# Autodesk Inventor assembly: 3000_Sample Assembly_V2
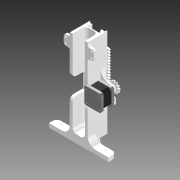
[picture p0: Inventor's stored thumbnail of the model, 180x180]
Saved by Autodesk Inventor 2021 (Build 250183000, 183)
## iProperties
Created: 2019-11-07
Part Number: 3000_Sample Assembly_V2
Document SubType Name: Assembly
Designer: RFLab
Author: RFLab
## Documents named in this file (7)
- C:\Users\RFLab\Documents\GitHub\MPS\Inventor Parts\MPSV2\6xxx_Sample Assembly\6000_Sample Assembly_V2.iam
- C:\Users\RFLab\Documents\GitHub\MPS\Inventor Parts\MPSV2\6xxx_Sample Assembly\61xx_Sample Rails\6101_Sample Rail Base_V2.ipt
- C:\Users\RFLab\Documents\GitHub\MPS\Inventor Parts\MPSV2\6xxx_Sample Assembly\61xx_Sample Rails\6102_Dovetail Slider_V2.ipt
- C:\Users\RFLab\Documents\GitHub\MPS\Inventor Parts\MPSV2\6xxx_Sample Assembly\62xx_ Motor and Driving\621x_Stepper Motor Parts\6211_Stepper Motor_V1.ipt
- C:\Users\RFLab\Documents\GitHub\MPS\Inventor Parts\MPSV2\6xxx_Sample Assembly\62xx_ Motor and Driving\622x_Motor Mechanical Connectors\6221_Motor Pinion_V3.ipt
- C:\Users\RFLab\Documents\GitHub\MPS\Inventor Parts\MPSV2\6xxx_Sample Assembly\61xx_Sample Rails\6104_Example Bulb_V1.ipt
- C:\Users\RFLab\Documents\GitHub\MPS\Inventor Parts\MPSV2\6xxx_Sample Assembly\61xx_Sample Rails\6103_Bulb Arm_V4.ipt
## Components (6 placed, 6 different names)
1. 6101_Sample Rail Base_V2:1 — Mate:1, Mate:2, Mate:13, Mate:14, Mate:15, Flush:3, Mate:17, Flush:4
2. 6102_Dovetail Slider_V2:1 — Mate:1, Mate:2, Mate:23, Flush:5, Mate:24
3. 6211_Stepper Motor_V1:1 — Flush:3, Mate:17, Flush:4, Rotational:1
4. Spur Gear1:2 — Rotational:1
5. 6104_Example Bulb_V1:1 — Mate:25, Mate:26
6. 6103_Bulb Arm_V4:1 — Mate:23, Flush:5, Mate:24, Mate:25, Mate:26
## Relationships (14: Mate 10, Flush 3, RevoluteJoint 1)
- Mate:1: 6101_Sample Rail Base_V2:1 ↔ 6102_Dovetail Slider_V2:1
- Mate:2 (-0.3 mm): 6101_Sample Rail Base_V2:1 ↔ 6102_Dovetail Slider_V2:1
- Mate:13: 6101_Sample Rail Base_V2:1
- Mate:14: 6101_Sample Rail Base_V2:1
- Mate:15: 6101_Sample Rail Base_V2:1
- Flush:3: 6101_Sample Rail Base_V2:1 ↔ 6211_Stepper Motor_V1:1
- Mate:17: 6101_Sample Rail Base_V2:1 ↔ 6211_Stepper Motor_V1:1
- Flush:4: 6101_Sample Rail Base_V2:1 ↔ 6211_Stepper Motor_V1:1
- Mate:23: 6102_Dovetail Slider_V2:1 ↔ 6103_Bulb Arm_V4:1
- Flush:5: 6102_Dovetail Slider_V2:1 ↔ 6103_Bulb Arm_V4:1
- Mate:24: 6102_Dovetail Slider_V2:1 ↔ 6103_Bulb Arm_V4:1
- Mate:25: 6104_Example Bulb_V1:1 ↔ 6103_Bulb Arm_V4:1
- Mate:26 (-2 mm): 6104_Example Bulb_V1:1 ↔ 6103_Bulb Arm_V4:1
- Rotational:1 [RevoluteJoint]: 6211_Stepper Motor_V1:1 ↔ Spur Gear1:2
